# Autodesk Inventor assembly: Output Shaft
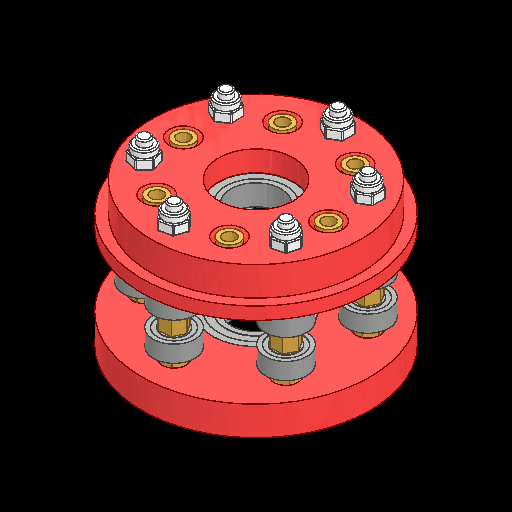
[picture p0: Inventor's stored thumbnail of the model, 512x512]
Saved by Autodesk Inventor 2025.2 (Build 292293000, 293)
## iProperties
Created: 2026-08-17
Part Number: Output Shaft
Document SubType Name: Assembly
Designer: valer
Author: valer
## Documents named in this file (9)
- C:\Users\valer\Desktop\Cycloidal-BDLC\parts\Output Shaft.iam
- C:\Users\valer\Desktop\Cycloidal-BDLC\parts\Bottom Shaft.ipt
- C:\Users\valer\Desktop\Cycloidal-BDLC\parts\12x21x5mm Bearing.ipt
- C:\Users\valer\Desktop\Cycloidal-BDLC\parts\M3x40mm Screw.ipt
- C:\Users\valer\Desktop\Cycloidal-BDLC\parts\Top Shaft.ipt
- C:\Users\valer\Desktop\Cycloidal-BDLC\parts\M3x5 Standoff.ipt
- C:\Users\valer\Desktop\Cycloidal-BDLC\parts\3x10x4mm Bearing.ipt
- C:\Users\valer\Desktop\Cycloidal-BDLC\parts\M3_Locknut.ipt
- C:\Users\valer\Desktop\Cycloidal-BDLC\parts\M3x6mm Insert.ipt
## Components (46 placed, 8 different names)
1. Bottom Shaft:1 — Mate:1, Mate:2, Mate:3, Mate:4, Mate:5, Mate:6, Mate:7, Mate:8, Mate:9, Mate:10, Mate:11, Mate:12, Mate:13, Mate:14, Mate:15, Mate:16, Flush:1, Mate:18, Mate:23, Mate:25, Mate:27, Mate:29, Mate:31, Mate:33
2. 12x21x5mm Bearing:1 — Mate:3, Mate:4, Mate:17
3. M3x40mm Screw:1 — Mate:5, Mate:6, Mate:26, Mate:40, Mate:46, Mate:64, Mate:66
4. M3x40mm Screw:2 — Mate:15, Mate:16, Mate:24, Mate:41, Mate:42, Mate:62, Mate:68
5. M3x40mm Screw:3 — Mate:13, Mate:14, Mate:19, Mate:22, Mate:39, Mate:44, Mate:60, Mate:72
6. M3x40mm Screw:4 — Mate:11, Mate:12, Mate:32, Mate:38, Mate:52, Mate:58, Mate:74
7. M3x40mm Screw:5 — Mate:9, Mate:10, Mate:30, Mate:36, Mate:50, Mate:56, Mate:76
8. M3x40mm Screw:6 — Mate:7, Mate:8, Mate:28, Mate:34, Mate:48, Mate:54, Mate:70
9. Top Shaft:1 — Mate:17, Mate:18, Mate:19, Mate:20, Mate:21, Mate:67, Mate:69, Mate:71, Mate:73, Mate:75, Mate:77, Mate:78, Flush:6, Mate:79, Flush:7, Mate:80, Flush:8, Mate:81, Flush:9, Mate:82, Flush:10, Mate:83, Flush:11
10. 12x21x5mm Bearing:2 — Mate:20, Mate:21
11. M3x5 Standoff:1 — Mate:30, Mate:31, Mate:37
12. M3x5 Standoff:2 — Mate:22, Mate:23
13. M3x5 Standoff:3 — Mate:24, Mate:25
14. M3x5 Standoff:4 — Mate:32, Mate:33
15. M3x5 Standoff:5 — Mate:28, Mate:29, Mate:35
16. M3x5 Standoff:6 — Mate:26, Mate:27
17. 3x10x4mm Bearing:1 — Mate:34, Mate:35, Flush:4, Mate:49
18. 3x10x4mm Bearing:2 — Mate:36, Mate:37, Flush:2, Mate:51
19. 3x10x4mm Bearing:3 — Mate:38, Flush:2, Flush:3, Mate:53
20. 3x10x4mm Bearing:4 — Mate:41, Flush:5, Mate:43
21. 3x10x4mm Bearing:5 — Mate:40, Flush:4, Flush:5, Mate:47
22. 3x10x4mm Bearing:6 — Mate:39, Flush:3, Mate:45
23. M3x5 Standoff:7 — Mate:42, Mate:43, Mate:63
24. M3x5 Standoff:8 — Mate:44, Mate:45, Mate:61
25. M3x5 Standoff:9 — Mate:46, Mate:47, Mate:65
26. M3x5 Standoff:10 — Mate:48, Mate:49, Mate:55
27. M3x5 Standoff:11 — Mate:50, Mate:51, Mate:57
28. M3x5 Standoff:12 — Mate:52, Mate:53, Mate:59
29. 3x10x4mm Bearing:7 — Mate:54, Mate:55
30. 3x10x4mm Bearing:8 — Mate:56, Mate:57
31. 3x10x4mm Bearing:9 — Mate:58, Mate:59
32. 3x10x4mm Bearing:10 — Mate:60, Mate:61
33. 3x10x4mm Bearing:11 — Mate:62, Mate:63
34. 3x10x4mm Bearing:12 — Mate:64, Mate:65
35. M3_Locknut:1 — Mate:66, Mate:67
36. M3_Locknut:2 — Mate:68, Mate:69
37. M3_Locknut:3 — Mate:70, Mate:71
38. M3_Locknut:4 — Mate:72, Mate:73
39. M3_Locknut:5 — Mate:76, Mate:77
40. M3_Locknut:6 — Mate:74, Mate:75
41. M3x6mm Insert:1 — Mate:78, Flush:6
42. M3x6mm Insert:2 — Mate:79, Flush:7
43. M3x6mm Insert:3 — Mate:80, Flush:8
44. M3x6mm Insert:4 — Mate:81, Flush:9
45. M3x6mm Insert:5 — Mate:82, Flush:10
46. M3x6mm Insert:6 — Mate:83, Flush:11
## Relationships (94: Mate 83, Flush 11)
- Mate:1: Bottom Shaft:1
- Mate:2: Bottom Shaft:1
- Mate:3: Bottom Shaft:1 ↔ 12x21x5mm Bearing:1
- Mate:4: Bottom Shaft:1 ↔ 12x21x5mm Bearing:1
- Mate:5: Bottom Shaft:1 ↔ M3x40mm Screw:1
- Mate:6: Bottom Shaft:1 ↔ M3x40mm Screw:1
- Mate:7: Bottom Shaft:1 ↔ M3x40mm Screw:6
- Mate:8: Bottom Shaft:1 ↔ M3x40mm Screw:6
- Mate:9: Bottom Shaft:1 ↔ M3x40mm Screw:5
- Mate:10: Bottom Shaft:1 ↔ M3x40mm Screw:5
- Mate:11: Bottom Shaft:1 ↔ M3x40mm Screw:4
- Mate:12: Bottom Shaft:1 ↔ M3x40mm Screw:4
- Mate:13: Bottom Shaft:1 ↔ M3x40mm Screw:3
- Mate:14: Bottom Shaft:1 ↔ M3x40mm Screw:3
- Mate:15: Bottom Shaft:1 ↔ M3x40mm Screw:2
- Mate:16: Bottom Shaft:1 ↔ M3x40mm Screw:2
- Flush:1: Bottom Shaft:1
- Mate:17: 12x21x5mm Bearing:1 ↔ Top Shaft:1
- Mate:18 (17.5 mm): Bottom Shaft:1 ↔ Top Shaft:1
- Mate:19: M3x40mm Screw:3 ↔ Top Shaft:1
- Mate:20: Top Shaft:1 ↔ 12x21x5mm Bearing:2
- Mate:21: Top Shaft:1 ↔ 12x21x5mm Bearing:2
- Mate:22: M3x40mm Screw:3 ↔ M3x5 Standoff:2
- Mate:23: Bottom Shaft:1 ↔ M3x5 Standoff:2
- Mate:24: M3x40mm Screw:2 ↔ M3x5 Standoff:3
- Mate:25: Bottom Shaft:1 ↔ M3x5 Standoff:3
- Mate:26: M3x40mm Screw:1 ↔ M3x5 Standoff:6
- Mate:27: Bottom Shaft:1 ↔ M3x5 Standoff:6
- Mate:28: M3x40mm Screw:6 ↔ M3x5 Standoff:5
- Mate:29: Bottom Shaft:1 ↔ M3x5 Standoff:5
- Mate:30: M3x40mm Screw:5 ↔ M3x5 Standoff:1
- Mate:31: Bottom Shaft:1 ↔ M3x5 Standoff:1
- Mate:32: M3x40mm Screw:4 ↔ M3x5 Standoff:4
- Mate:33: Bottom Shaft:1 ↔ M3x5 Standoff:4
- Mate:34: M3x40mm Screw:6 ↔ 3x10x4mm Bearing:1
- Mate:35: M3x5 Standoff:5 ↔ 3x10x4mm Bearing:1
- Mate:36: M3x40mm Screw:5 ↔ 3x10x4mm Bearing:2
- Mate:37: M3x5 Standoff:1 ↔ 3x10x4mm Bearing:2
- Mate:38: M3x40mm Screw:4 ↔ 3x10x4mm Bearing:3
- Flush:2: 3x10x4mm Bearing:2 ↔ 3x10x4mm Bearing:3
- Mate:39: M3x40mm Screw:3 ↔ 3x10x4mm Bearing:6
- Flush:3: 3x10x4mm Bearing:3 ↔ 3x10x4mm Bearing:6
- Mate:40: M3x40mm Screw:1 ↔ 3x10x4mm Bearing:5
- Flush:4: 3x10x4mm Bearing:1 ↔ 3x10x4mm Bearing:5
- Mate:41: M3x40mm Screw:2 ↔ 3x10x4mm Bearing:4
- Flush:5: 3x10x4mm Bearing:4 ↔ 3x10x4mm Bearing:5
- Mate:42: M3x40mm Screw:2 ↔ M3x5 Standoff:7
- Mate:43: 3x10x4mm Bearing:4 ↔ M3x5 Standoff:7
- Mate:44: M3x40mm Screw:3 ↔ M3x5 Standoff:8
- Mate:45: 3x10x4mm Bearing:6 ↔ M3x5 Standoff:8
- Mate:46: M3x40mm Screw:1 ↔ M3x5 Standoff:9
- Mate:47: 3x10x4mm Bearing:5 ↔ M3x5 Standoff:9
- Mate:48: M3x40mm Screw:6 ↔ M3x5 Standoff:10
- Mate:49: 3x10x4mm Bearing:1 ↔ M3x5 Standoff:10
- Mate:50: M3x40mm Screw:5 ↔ M3x5 Standoff:11
- Mate:51: 3x10x4mm Bearing:2 ↔ M3x5 Standoff:11
- Mate:52: M3x40mm Screw:4 ↔ M3x5 Standoff:12
- Mate:53: 3x10x4mm Bearing:3 ↔ M3x5 Standoff:12
- Mate:54: M3x40mm Screw:6 ↔ 3x10x4mm Bearing:7
- Mate:55: M3x5 Standoff:10 ↔ 3x10x4mm Bearing:7
- Mate:56: M3x40mm Screw:5 ↔ 3x10x4mm Bearing:8
- Mate:57: M3x5 Standoff:11 ↔ 3x10x4mm Bearing:8
- Mate:58: M3x40mm Screw:4 ↔ 3x10x4mm Bearing:9
- Mate:59: M3x5 Standoff:12 ↔ 3x10x4mm Bearing:9
- Mate:60: M3x40mm Screw:3 ↔ 3x10x4mm Bearing:10
- Mate:61: M3x5 Standoff:8 ↔ 3x10x4mm Bearing:10
- Mate:62: M3x40mm Screw:2 ↔ 3x10x4mm Bearing:11
- Mate:63: M3x5 Standoff:7 ↔ 3x10x4mm Bearing:11
- Mate:64: M3x40mm Screw:1 ↔ 3x10x4mm Bearing:12
- Mate:65: M3x5 Standoff:9 ↔ 3x10x4mm Bearing:12
- Mate:66: M3x40mm Screw:1 ↔ M3_Locknut:1
- Mate:67: Top Shaft:1 ↔ M3_Locknut:1
- Mate:68: M3x40mm Screw:2 ↔ M3_Locknut:2
- Mate:69: Top Shaft:1 ↔ M3_Locknut:2
- Mate:70: M3x40mm Screw:6 ↔ M3_Locknut:3
- Mate:71: Top Shaft:1 ↔ M3_Locknut:3
- Mate:72: M3x40mm Screw:3 ↔ M3_Locknut:4
- Mate:73: Top Shaft:1 ↔ M3_Locknut:4
- Mate:74: M3x40mm Screw:4 ↔ M3_Locknut:6
- Mate:75: Top Shaft:1 ↔ M3_Locknut:6
- Mate:76: M3x40mm Screw:5 ↔ M3_Locknut:5
- Mate:77: Top Shaft:1 ↔ M3_Locknut:5
- Mate:78: Top Shaft:1 ↔ M3x6mm Insert:1
- Flush:6: Top Shaft:1 ↔ M3x6mm Insert:1
- Mate:79: Top Shaft:1 ↔ M3x6mm Insert:2
- Flush:7: Top Shaft:1 ↔ M3x6mm Insert:2
- Mate:80: Top Shaft:1 ↔ M3x6mm Insert:3
- Flush:8: Top Shaft:1 ↔ M3x6mm Insert:3
- Mate:81: Top Shaft:1 ↔ M3x6mm Insert:4
- Flush:9: Top Shaft:1 ↔ M3x6mm Insert:4
- Mate:82: Top Shaft:1 ↔ M3x6mm Insert:5
- Flush:10: Top Shaft:1 ↔ M3x6mm Insert:5
- Mate:83: Top Shaft:1 ↔ M3x6mm Insert:6
- Flush:11: Top Shaft:1 ↔ M3x6mm Insert:6
